# Autodesk Inventor assembly: printer corner
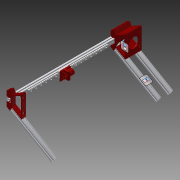
[picture p0: Inventor's stored thumbnail of the model, 180x180]
Saved by Autodesk Inventor 2015 SP1 (Build 190203100, 203)
## iProperties
Created: 2015-01-27
Part Number: printer corner
Document SubType Name: Assembly
Designer: Joseph
Author: Joseph
## Documents named in this file (6)
- C:\Users\Joseph\Documents\GitHub\mchp_kossel\Printer\printer corner.iam
- C:\Users\Joseph\Documents\GitHub\mchp_kossel\Printer\240 beam.ipt
- C:\Users\Joseph\Documents\GitHub\mchp_kossel\Printer\lower corner.ipt
- C:\Users\Joseph\Documents\GitHub\mchp_kossel\Printer\600 beam.ipt
- C:\Users\Joseph\Documents\GitHub\mchp_kossel\Printer\linear slide.iam
- C:\Users\Joseph\Documents\GitHub\mchp_kossel\Printer\top corner.ipt
## Components (7 placed, 5 different names)
1. 240 beam:3 — Mate:50, Flush:17, Flush:19, Mate:51
2. 240 beam:4 — Flush:17, Flush:18, Mate:52
3. lower corner:3 — Mate:50, Flush:18, Flush:19, Mate:51, Mate:52, Flush:20, Mate:53, Flush:23
4. 600 beam:1 — Flush:20, Mate:53, Flush:22, Mate:54, Mate:55, Flush:23, Mate:58
5. linear slide:1 [sub-assembly] — Mate:58
6. 240 beam:5 — Flush:21, Mate:56, Mate:57
7. top corner:1 — Flush:21, Flush:22, Mate:54, Mate:55, Mate:56, Mate:57
## Relationships (16: Mate 9, Flush 7)
- Mate:50: 240 beam:3 ↔ lower corner:3
- Flush:17: 240 beam:3 ↔ 240 beam:4
- Flush:18: 240 beam:4 ↔ lower corner:3
- Flush:19: 240 beam:3 ↔ lower corner:3
- Mate:51: 240 beam:3 ↔ lower corner:3
- Mate:52: 240 beam:4 ↔ lower corner:3
- Flush:20: lower corner:3 ↔ 600 beam:1
- Mate:53: lower corner:3 ↔ 600 beam:1
- Flush:21: 240 beam:5 ↔ top corner:1
- Flush:22: 600 beam:1 ↔ top corner:1
- Mate:54: 600 beam:1 ↔ top corner:1
- Mate:55: 600 beam:1 ↔ top corner:1
- Mate:56: 240 beam:5 ↔ top corner:1
- Mate:57: 240 beam:5 ↔ top corner:1
- Flush:23: lower corner:3 ↔ 600 beam:1
- Mate:58: 600 beam:1 ↔ linear slide:1
